# Autodesk Inventor assembly: tether-assembly
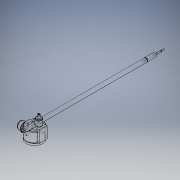
[picture p0: Inventor's stored thumbnail of the model, 180x180]
Saved by Autodesk Inventor 2019 (Build 230136000, 136)
## iProperties
Created: 2019-05-18
Part Number: tether-assembly
Document SubType Name: Assembly
Designer: Wilson Lab
Author: Wilson Lab
## Documents named in this file (6)
- C:\code\auditory-behavior-experiments\design-files\tether-assembly\tether-assembly.iam
- C:\code\auditory-behavior-experiments\design-files\tether-assembly\ER8-Solidworks.ipt
- C:\code\auditory-behavior-experiments\design-files\tether-assembly\pin_adapter.ipt
- C:\code\auditory-behavior-experiments\design-files\tether-assembly\female_pin_component.ipt
- C:\code\auditory-behavior-experiments\design-files\tether-assembly\male_pin_component.ipt
- C:\code\auditory-behavior-experiments\design-files\vr-opto-assembly\91240000E_step.ipt
## Components (5 placed, 5 different names)
1. ER8-Solidworks:1 — Rigid:1, Mate:1, Tangent:1
2. pin_adapter:1 — Rigid:1, Rigid:2
3. female_pin_component:1 — Rigid:2, Rigid:3
4. male_pin_component:1 — Rigid:3
5. 91240000E_step:1 — Mate:1, Tangent:1, Mate:2, Mate:3
## Relationships (7: WeldJoint 3, Mate 3, Tangent 1)
- Rigid:1 [WeldJoint]: ER8-Solidworks:1 ↔ pin_adapter:1
- Rigid:2 [WeldJoint]: pin_adapter:1 ↔ female_pin_component:1
- Rigid:3 [WeldJoint]: female_pin_component:1 ↔ male_pin_component:1
- Mate:1 (-25.4 mm): ER8-Solidworks:1 ↔ 91240000E_step:1
- Tangent:1 (-4.445 mm): ER8-Solidworks:1 ↔ 91240000E_step:1
- Mate:2: 91240000E_step:1
- Mate:3: 91240000E_step:1
